# Autodesk Inventor assembly: eye ass
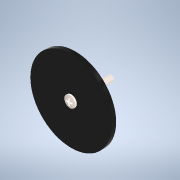
[picture p0: Inventor's stored thumbnail of the model, 180x180]
Saved by Autodesk Inventor 2021 (Build 250183000, 183)
## iProperties
Created: 2023-06-07
Part Number: eye ass
Document SubType Name: Assembly
Designer: shrus
Author: shrus
## Documents named in this file (3)
- C:\Users\shrus\Documents\eye ass.iam
- C:\Users\shrus\Documents\eye.ipt
- C:\Users\shrus\Documents\m3-6mm.ipt
## Components (2 placed, 2 different names)
1. Part6:1 — Mate:1
2. m3-6mm:1 — Mate:1
## Relationships (1: Mate 1)
- Mate:1: Part6:1 ↔ m3-6mm:1
